# Autodesk Inventor assembly: photoTransistorAssembly
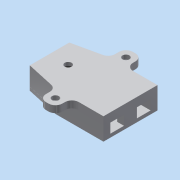
[picture p0: Inventor's stored thumbnail of the model, 180x180]
Saved by Autodesk Inventor 2017 (Build 210142000, 142)
## iProperties
Created: 2016-12-12
Part Number: photoTransistorAssembly
Document SubType Name: Assembly
Designer: techn
Author: techn
## Documents named in this file (4)
- D:\OneDrive\Documents\Other Projects\Submarine\CAD\aft\encoder\photoTransistorAssembly.iam
- D:\OneDrive\Documents\Other Projects\Submarine\CAD\aft\encoder\photoTransistor.ipt
- D:\OneDrive\Documents\Other Projects\Submarine\CAD\aft\encoder\phototransistorMount1.ipt
- D:\OneDrive\Documents\Other Projects\Submarine\CAD\aft\encoder\phototransistorMount2.ipt
## Components (3 placed, 3 different names)
1. photoTransistor:1 — Mate:1, Mate:3, Flush:1
2. phototransistorMount1:1 — Mate:1, Mate:2, Mate:3, Flush:1, Flush:2, Flush:3
3. phototransistorMount2:1 — Mate:2, Flush:2, Flush:3
## Relationships (6: Mate 3, Flush 3)
- Mate:1 (0.635 mm): photoTransistor:1 ↔ phototransistorMount1:1
- Mate:2: phototransistorMount1:1 ↔ phototransistorMount2:1
- Mate:3: photoTransistor:1 ↔ phototransistorMount1:1
- Flush:1: photoTransistor:1 ↔ phototransistorMount1:1
- Flush:2: phototransistorMount1:1 ↔ phototransistorMount2:1
- Flush:3: phototransistorMount1:1 ↔ phototransistorMount2:1
